# Autodesk Inventor assembly: hotplateassembly
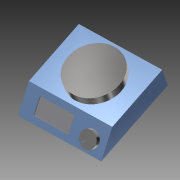
[picture p0: Inventor's stored thumbnail of the model, 180x180]
Saved by Autodesk Inventor 2014 (Build 180170000, 170)
## iProperties
Created: 2014-07-17
Part Number: hotplateassembly
Document SubType Name: Assembly
Designer: Nabeel
Author: Nabeel
## Documents named in this file (4)
- C:\Users\Nabeel\Desktop\Shielding\Project\Assets\NPRE 100 Laboratory\Calorimeter\Hotplate\hotplateassembly.iam
- C:\Users\Nabeel\Desktop\Shielding\Project\Assets\NPRE 100 Laboratory\Calorimeter\Hotplate\hotbody.ipt
- C:\Users\Nabeel\Desktop\Shielding\Project\Assets\NPRE 100 Laboratory\Calorimeter\Hotplate\hotbuton.ipt
- C:\Users\Nabeel\Desktop\Shielding\Project\Assets\NPRE 100 Laboratory\Calorimeter\Hotplate\hottop.ipt
## Components (3 placed, 3 different names)
1. hotbody:1 — Mate:1, Mate:2
2. hotbuton:1 — Mate:1
3. hottop:1 — Mate:2
## Relationships (2: Mate 2)
- Mate:1: hotbody:1 ↔ hotbuton:1
- Mate:2: hotbody:1 ↔ hottop:1
